# Autodesk Inventor assembly: 12V 350RPM Small DFRobot Motor v8
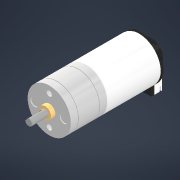
[picture p0: Inventor's stored thumbnail of the model, 180x180]
Saved by Autodesk Inventor 2021 (Build 250183000, 183)
## iProperties
Created: 2021-08-11
Part Number: 12V 350RPM Small DFRobot Motor v8
Document SubType Name: Assembly
Designer: rocke
Sending System: Autodesk Translation Framework v10.9.0.1377
Preprocessor: ST-DEVELOPER v18.1
Title: C:/Users/Jacob/Google Drive/Documents/3D Printing/3D Downloads/For Thingiverse Publishing/DFRobot 12V 350RPM Small Motor/12V 350RPM Small DFRobot Motor v8.step
## Documents named in this file (9)
- C:\Users\rocke\Downloads\12V 350RPM Small DFRobot Motor v8.iam
- C:\Users\rocke\Downloads\Shaft.ipt
- C:\Users\rocke\Downloads\Shaft_Coller.ipt
- C:\Users\rocke\Downloads\Body_Back.ipt
- C:\Users\rocke\Downloads\Body_Front.ipt
- C:\Users\rocke\Downloads\B6B-XH-AM v6.iam
- C:\Users\rocke\Downloads\PCB.ipt
- C:\Users\rocke\Downloads\EncoderMagnet.ipt
- C:\Users\rocke\Downloads\Text.ipt
## Components (8 placed, 8 different names)
1. Shaft:1 — Rotational:1
2. Shaft_Coller:1 — Rotational:1
3. Body_Back:1
4. Body_Front:1
5. B6B-XH-AM v6:1 [sub-assembly]
6. PCB:1
7. EncoderMagnet:1
8. Text:1
## Relationships (1: RevoluteJoint 1)
- Rotational:1 [RevoluteJoint] (1.5 mm): Shaft:1 ↔ Shaft_Coller:1
